# Autodesk Inventor assembly: Tube Replacements
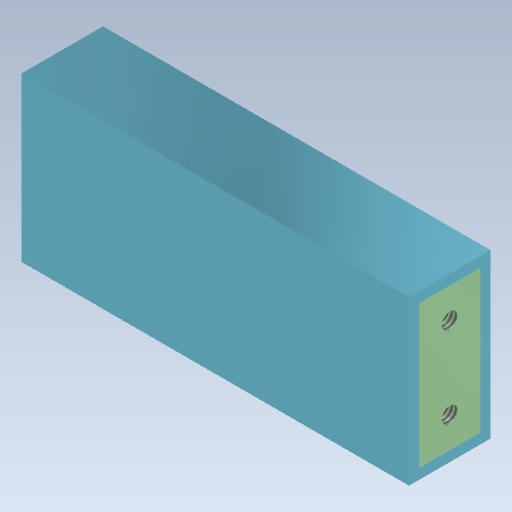
[picture p0: Inventor's stored thumbnail of the model, 512x512]
Saved by Autodesk Inventor 2020 (Build 240168000, 168)
## iProperties
Created: 2019-09-11
Part Number: Tube Replacements
Document SubType Name: Assembly
Designer: Matt
Author: Matt
## Documents named in this file (3)
- C:\Users\mpark\Documents\NASA20\Inventor Files\NASA-20\NASA-20\Tube Replacements.iam
- C:\Users\mpark\Documents\NASA20\Inventor Files\NASA-20\NASA-20\SQ Tube.ipt
- C:\Users\mpark\Documents\NASA20\Inventor Files\NASA-20\NASA-20\Threaded Block.ipt
## Components (2 placed, 2 different names)
1. SQ Tube:1 — Mate:1, Mate:2, Flush:1
2. Threaded Block:1 — Mate:1, Mate:2, Flush:1
## Relationships (3: Mate 2, Flush 1)
- Mate:1: SQ Tube:1 ↔ Threaded Block:1
- Mate:2: SQ Tube:1 ↔ Threaded Block:1
- Flush:1: SQ Tube:1 ↔ Threaded Block:1
